# Autodesk Inventor assembly: SPE0V1 Ensamble General
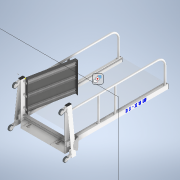
[picture p0: Inventor's stored thumbnail of the model, 180x180]
Saved by Autodesk Inventor 2021.2 (Build 252289000, 289)
## iProperties
Created: 2026-05-12
Part Number: SPE0V1 Ensamble General
Document SubType Name: Assembly
Designer: nelso
Author: nelso
## Documents named in this file (19)
- C:\Users\nelso\Desktop\Soporte-Paciente-Espinografia\Workspace\SPE0V1 Ensamble General.iam
- C:\Users\nelso\Desktop\Soporte-Paciente-Espinografia\Workspace\SP25V1 Acrilico.ipt
- C:\Users\nelso\Desktop\Soporte-Paciente-Espinografia\Workspace\SPE1V1 Estructura.iam
- C:\Users\nelso\Desktop\Soporte-Paciente-Espinografia\Workspace\SPE2V1 Baranda.iam
- C:\Users\nelso\Desktop\Soporte-Paciente-Espinografia\Workspace\DIN933M8X1.25L20C.ipt
- C:\Users\nelso\Desktop\Soporte-Paciente-Espinografia\Workspace\DIN125-A8,4C.ipt
- C:\Users\nelso\Desktop\Soporte-Paciente-Espinografia\Workspace\Logo.ipt
- C:\Users\nelso\Desktop\Soporte-Paciente-Espinografia\Workspace\SP28V1 Seguro Acrilico.ipt
- C:\Users\nelso\Desktop\Soporte-Paciente-Espinografia\Workspace\SP26V1 Base Chapa.ipt
- C:\Users\nelso\Desktop\Soporte-Paciente-Espinografia\Workspace\SP32V1 Refuerzo.ipt
- C:\Users\nelso\Desktop\Soporte-Paciente-Espinografia\Workspace\SPE31V1 Bisagra.iam
- C:\Users\nelso\Desktop\Soporte-Paciente-Espinografia\Workspace\SP39V1 Chapa Acrilico.ipt
- C:\Users\nelso\Desktop\Soporte-Paciente-Espinografia\Workspace\ISO7380M4X0.8L16I.ipt
- C:\Users\nelso\Desktop\Soporte-Paciente-Espinografia\Workspace\DIN555-5M4X0.8I.ipt
- C:\Users\nelso\Desktop\Soporte-Paciente-Espinografia\Workspace\SPE37V1 Cierre Superior.iam
- C:\Users\nelso\Desktop\Soporte-Paciente-Espinografia\Workspace\DIN125A4C.ipt
- C:\Users\nelso\Desktop\Soporte-Paciente-Espinografia\Workspace\DIN 555A5C.ipt
- C:\Users\nelso\Desktop\Soporte-Paciente-Espinografia\Workspace\DIN125-A6C.ipt
- C:\Users\nelso\Desktop\Soporte-Paciente-Espinografia\Workspace\DIN912-M6X1L16P.ipt
## Components (140 placed, 18 different names)
1. SP26V1 Base Chapa:1 — Mate:343, Mate:344, Mate:345, Mate:346, Mate:347, Mate:348, Mate:350, Mate:351, Mate:352, Mate:353, Mate:354, Flush:49, Flush:50, Flush:51, Angle:1, Mate:500, Mate:501, Mate:502, Mate:503, Mate:504, Mate:505
2. SP25V1 Acrilico:1 — Mate:179, Mate:180, Flush:19, Flush:20, Mate:262, Mate:355, Mate:356, Mate:357, Flush:52, Flush:53
3. SPE1V1 Estructura:1 [sub-assembly] — Coincidencia:100, Coincidencia:101, Coincidencia:102, Coincidencia:117, Nivelación:14, Nivelación:15, Mate:235, Mate:236, Mate:237, Flush:40, Mate:239, Mate:240, Mate:241, Flush:42, Mate:324, Mate:325, Flush:47, Flush:48, Mate:331, Mate:332, Mate:333, Mate:337, Mate:338, Mate:339, Mate:340, Mate:341, Mate:342, Angle:1, Flush:52, Mate:451, Mate:513, Mate:514, Mate:516, Mate:517, Mate:524, Mate:526
4. SPE2V1 Baranda:2 [sub-assembly] — Coincidencia:100, Coincidencia:101, Coincidencia:102, Coincidencia:109, Coincidencia:110, Coincidencia:111, Coincidencia:112, Mate:134, Mate:135, Mate:136, Mate:137, Mate:138, Mate:139, Mate:140, Mate:141, Mate:142, Mate:143, Mate:144, Mate:145, Mate:168, Mate:169, Mate:170, Mate:171, Mate:172, Mate:173
5. SPE2V1 Baranda:3 [sub-assembly] — Mate:118, Mate:119, Mate:120, Mate:121, Mate:122, Mate:123, Mate:124, Mate:125, Mate:126, Mate:127, Mate:128, Mate:129, Mate:130, Mate:131, Mate:132, Mate:133, Mate:147, Mate:149, Mate:156, Mate:157, Mate:158, Mate:159, Mate:160, Mate:161, Mate:235, Mate:236
6. DIN933M8X1.25L20C:1 — Coincidencia:113, Coincidencia:114
7. DIN125-A8,4C:1 — Coincidencia:109, Coincidencia:110, Coincidencia:115, Coincidencia:116
8. DIN125-A8,4C:2 — Coincidencia:111, Coincidencia:112, Coincidencia:113, Coincidencia:114
9. DIN933M8X1.25L20C:2 — Coincidencia:115, Coincidencia:116
10. Logo:1 — Coincidencia:117, Nivelación:14, Nivelación:15
11. DIN125-A8,4C:3 — Mate:144, Mate:145, Mate:162
12. DIN125-A8,4C:4 — Mate:142, Mate:143, Mate:163
13. DIN125-A8,4C:5 — Mate:140, Mate:141, Mate:164
14. DIN125-A8,4C:6 — Mate:138, Mate:139, Mate:165
15. DIN125-A8,4C:7 — Mate:135, Mate:136, Mate:167
16. DIN125-A8,4C:8 — Mate:134, Mate:137, Mate:166
17. DIN125-A8,4C:9 — Mate:130, Mate:132, Mate:155
18. DIN125-A8,4C:10 — Mate:131, Mate:133, Mate:154
19. DIN125-A8,4C:11 — Mate:128, Mate:129, Mate:153
20. DIN125-A8,4C:12 — Mate:126, Mate:127, Mate:152
21. DIN125-A8,4C:13 — Mate:122, Mate:123, Mate:150
22. DIN125-A8,4C:14 — Mate:124, Mate:125, Mate:151
23. DIN125-A8,4C:15 — Mate:120, Mate:121, Mate:148
24. DIN125-A8,4C:16 — Mate:118, Mate:119, Mate:146
25. DIN933M8X1.25L20C:3 — Mate:162, Mate:168
26. DIN933M8X1.25L20C:4 — Mate:163, Mate:169
27. DIN933M8X1.25L20C:5 — Mate:164, Mate:170
28. DIN933M8X1.25L20C:6 — Mate:165, Mate:171
29. DIN933M8X1.25L20C:7 — Mate:166, Mate:172
30. DIN933M8X1.25L20C:8 — Mate:167, Mate:173
31. DIN933M8X1.25L20C:9 — Mate:155, Mate:156
32. DIN933M8X1.25L20C:10 — Mate:154, Mate:157
33. DIN933M8X1.25L20C:11 — Mate:153, Mate:159
34. DIN933M8X1.25L20C:12 — Mate:152, Mate:158
35. DIN933M8X1.25L20C:13 — Mate:151, Mate:160
36. DIN933M8X1.25L20C:14 — Mate:150, Mate:161, Mate:237
37. DIN933M8X1.25L20C:15 — Mate:148, Mate:149
38. DIN933M8X1.25L20C:16 — Mate:146, Mate:147
39. SP28V1 Seguro Acrilico:1 — Mate:179, Flush:19, Mate:199, Mate:200, Mate:201, Mate:202, Mate:203, Mate:204, Mate:205, Mate:206, Mate:207, Mate:217, Mate:218, Mate:219, Mate:220, Mate:221, Mate:222, Mate:223, Mate:224, Mate:225, Flush:53
40. SP28V1 Seguro Acrilico:2 — Mate:180, Flush:20, Mate:208, Mate:209, Mate:210, Mate:211, Mate:212, Mate:213, Mate:214, Mate:215, Mate:216, Mate:227, Mate:228, Mate:229, Mate:230, Mate:231, Mate:233, Flush:40, Flush:42, Mate:448, Mate:449, Mate:450
41. ISO7380M4X0.8L16I:1 — Mate:199, Mate:217, Mate:358, Mate:411
42. ISO7380M4X0.8L16I:2 — Mate:200, Mate:218, Mate:359, Mate:410
43. ISO7380M4X0.8L16I:3 — Mate:201, Mate:219, Mate:360, Mate:409
44. ISO7380M4X0.8L16I:4 — Mate:202, Mate:220, Mate:361, Mate:408
45. ISO7380M4X0.8L16I:5 — Mate:203, Mate:221, Mate:362, Mate:407
46. ISO7380M4X0.8L16I:6 — Mate:204, Mate:222, Mate:363, Mate:406
47. ISO7380M4X0.8L16I:7 — Mate:205, Mate:223, Mate:364, Mate:405
48. ISO7380M4X0.8L16I:8 — Mate:206, Mate:224, Mate:365, Mate:404
49. ISO7380M4X0.8L16I:9 — Mate:207, Mate:225, Mate:366, Mate:403
50. ISO7380M4X0.8L16I:10 — Mate:208, Mate:262, Mate:367, Mate:394, Mate:449
51. ISO7380M4X0.8L16I:11 — Mate:209, Mate:233, Mate:368, Mate:395
52. ISO7380M4X0.8L16I:12 — Mate:210, Mate:369, Mate:396, Mate:450
53. ISO7380M4X0.8L16I:13 — Mate:211, Mate:231, Mate:370, Mate:397
54. ISO7380M4X0.8L16I:14 — Mate:212, Mate:230, Mate:371, Mate:398
55. ISO7380M4X0.8L16I:15 — Mate:214, Mate:228, Mate:373, Mate:400
56. ISO7380M4X0.8L16I:16 — Mate:215, Mate:227, Mate:374, Mate:402
57. ISO7380M4X0.8L16I:17 — Mate:216, Mate:375, Mate:401, Mate:448
58. ISO7380M4X0.8L16I:18 — Mate:213, Mate:229, Mate:372, Mate:399
59. SP32V1 Refuerzo:1 — Mate:351, Mate:354, Flush:50
60. SP32V1 Refuerzo:2 — Mate:348, Mate:353, Flush:49
61. SP32V1 Refuerzo:3 — Mate:350, Mate:352, Flush:51
62. SPE31V1 Bisagra:1 [sub-assembly] — Mate:333, Mate:341, Mate:342, Mate:345, Mate:347, Mate:468, Mate:469, Mate:470, Mate:471, Mate:472, Mate:473, Mate:474, Mate:475
63. SPE31V1 Bisagra:2 [sub-assembly] — Mate:331, Mate:337, Mate:338, Mate:344, Mate:346, Mate:452, Mate:453, Mate:454, Mate:455, Mate:456, Mate:457, Mate:458, Mate:459
64. SPE31V1 Bisagra:3 [sub-assembly] — Mate:332, Mate:339, Mate:340, Mate:343, Mate:460, Mate:461, Mate:462, Mate:463, Mate:464, Mate:465, Mate:466, Mate:467
65. SP39V1 Chapa Acrilico:1 — Mate:325, Flush:47, Mate:355, Mate:430, Mate:432, Mate:434, Mate:436, Mate:438, Mate:440, Mate:442, Mate:444, Mate:446
66. SP39V1 Chapa Acrilico:2 — Mate:324, Flush:48, Mate:357, Mate:412, Mate:414, Mate:416, Mate:418, Mate:420, Mate:422, Mate:424, Mate:426, Mate:428
67. DIN555-5M4X0.8I:1 — Mate:358, Mate:413
68. DIN555-5M4X0.8I:2 — Mate:359, Mate:415
69. DIN555-5M4X0.8I:3 — Mate:360, Mate:417
70. DIN555-5M4X0.8I:4 — Mate:361, Mate:419
71. DIN555-5M4X0.8I:5 — Mate:362, Mate:421
72. DIN555-5M4X0.8I:6 — Mate:363, Mate:423
73. DIN555-5M4X0.8I:7 — Mate:364, Mate:425
74. DIN555-5M4X0.8I:8 — Mate:365, Mate:427
75. DIN555-5M4X0.8I:9 — Mate:366, Mate:429
76. DIN555-5M4X0.8I:10 — Mate:367, Mate:447
77. DIN555-5M4X0.8I:11 — Mate:368, Mate:445
78. DIN555-5M4X0.8I:12 — Mate:369, Mate:443
79. DIN555-5M4X0.8I:13 — Mate:370, Mate:441
80. DIN555-5M4X0.8I:14 — Mate:371, Mate:439
81. DIN555-5M4X0.8I:15 — Mate:372, Mate:437
82. DIN555-5M4X0.8I:16 — Mate:373, Mate:435
83. DIN555-5M4X0.8I:17 — Mate:374, Mate:433
84. DIN555-5M4X0.8I:18 — Mate:375, Mate:431
85. DIN125A4C:2 — Mate:411, Mate:412, Mate:413
86. DIN125A4C:3 — Mate:410, Mate:414, Mate:415
87. DIN125A4C:4 — Mate:409, Mate:416, Mate:417
88. DIN125A4C:5 — Mate:408, Mate:418, Mate:419
89. DIN125A4C:6 — Mate:407, Mate:420, Mate:421
90. DIN125A4C:7 — Mate:406, Mate:422, Mate:423
91. DIN125A4C:8 — Mate:405, Mate:424, Mate:425
92. DIN125A4C:9 — Mate:404, Mate:426, Mate:427
93. DIN125A4C:10 — Mate:403, Mate:428, Mate:429
94. DIN125A4C:11 — Mate:402, Mate:432, Mate:433
95. DIN125A4C:12 — Mate:401, Mate:430, Mate:431
96. DIN125A4C:13 — Mate:400, Mate:434, Mate:435
97. DIN125A4C:14 — Mate:399, Mate:436, Mate:437
98. DIN125A4C:15 — Mate:398, Mate:438, Mate:439
99. DIN125A4C:16 — Mate:397, Mate:440, Mate:441
100. DIN125A4C:17 — Mate:396, Mate:442, Mate:443
101. DIN125A4C:18 — Mate:395, Mate:444, Mate:445
102. DIN125A4C:19 — Mate:394, Mate:446, Mate:447
103. SPE37V1 Cierre Superior:1 [sub-assembly] — Mate:451
104. DIN912-M6X1L16P:2 — Mate:452, Mate:454, Mate:522
105. DIN912-M6X1L16P:3 — Mate:453, Mate:455, Mate:523, Mate:525
106. DIN912-M6X1L16P:4 — Mate:456, Mate:457, Mate:506
107. DIN912-M6X1L16P:5 — Mate:458, Mate:459, Mate:507
108. DIN912-M6X1L16P:6 — Mate:460, Mate:464, Mate:518
109. DIN912-M6X1L16P:7 — Mate:462, Mate:466, Mate:508
110. DIN912-M6X1L16P:8 — Mate:461, Mate:465, Mate:519
111. DIN912-M6X1L16P:9 — Mate:463, Mate:467, Mate:509
112. DIN912-M6X1L16P:10 — Mate:469, Mate:473, Mate:521
113. DIN912-M6X1L16P:11 — Mate:468, Mate:472, Mate:520
114. DIN912-M6X1L16P:12 — Mate:470, Mate:474, Mate:510
115. DIN912-M6X1L16P:13 — Mate:471, Mate:475, Mate:511
116. DIN 555A5C:1 — Mate:476, Mate:488, Mate:519
117. DIN 555A5C:2 — Mate:477, Mate:489, Mate:506
118. DIN 555A5C:3 — Mate:478, Mate:523
119. DIN 555A5C:4 — Mate:479, Mate:491, Mate:509
120. DIN 555A5C:5 — Mate:480, Mate:492, Mate:518
121. DIN 555A5C:6 — Mate:481, Mate:493, Mate:508
122. DIN 555A5C:7 — Mate:482, Mate:494, Mate:521
123. DIN 555A5C:8 — Mate:483, Mate:495, Mate:510
124. DIN 555A5C:9 — Mate:485, Mate:497, Mate:522
125. DIN 555A5C:10 — Mate:484, Mate:496, Mate:507
126. DIN 555A5C:11 — Mate:486, Mate:498, Mate:511
127. DIN 555A5C:12 — Mate:487, Mate:499, Mate:520
128. DIN125-A6C:1 — Mate:476, Mate:488, Mate:513
129. DIN125-A6C:2 — Mate:477, Mate:489, Mate:500
130. DIN125-A6C:3 — Mate:478, Mate:524, Mate:525
131. DIN125-A6C:4 — Mate:479, Mate:491, Mate:502
132. DIN125-A6C:5 — Mate:480, Mate:492, Mate:514
133. DIN125-A6C:6 — Mate:481, Mate:493, Mate:503
134. DIN125-A6C:7 — Mate:482, Mate:494, Mate:517
135. DIN125-A6C:8 — Mate:483, Mate:495, Mate:504
136. DIN125-A6C:9 — Mate:484, Mate:496, Mate:501
137. DIN125-A6C:10 — Mate:485, Mate:497, Mate:526
138. DIN125-A6C:11 — Mate:486, Mate:498, Mate:505
139. DIN125-A6C:12 — Mate:487, Mate:499, Mate:516
140. DIN912-M6X1L16P:1
## Relationships (297: Mate 283, Flush 13, Angle 1)
- Coincidencia:100 [Mate]: SPE1V1 Estructura:1 ↔ SPE2V1 Baranda:2
- Coincidencia:101 [Mate]: SPE1V1 Estructura:1 ↔ SPE2V1 Baranda:2
- Coincidencia:102 [Mate]: SPE1V1 Estructura:1 ↔ SPE2V1 Baranda:2
- Coincidencia:109 [Mate]: SPE2V1 Baranda:2 ↔ DIN125-A8,4C:1
- Coincidencia:110 [Mate]: SPE2V1 Baranda:2 ↔ DIN125-A8,4C:1
- Coincidencia:111 [Mate]: SPE2V1 Baranda:2 ↔ DIN125-A8,4C:2
- Coincidencia:112 [Mate]: SPE2V1 Baranda:2 ↔ DIN125-A8,4C:2
- Coincidencia:113 [Mate]: DIN933M8X1.25L20C:1 ↔ DIN125-A8,4C:2
- Coincidencia:114 [Mate]: DIN933M8X1.25L20C:1 ↔ DIN125-A8,4C:2
- Coincidencia:115 [Mate]: DIN125-A8,4C:1 ↔ DIN933M8X1.25L20C:2
- Coincidencia:116 [Mate]: DIN125-A8,4C:1 ↔ DIN933M8X1.25L20C:2
- Coincidencia:117 [Mate]: SPE1V1 Estructura:1 ↔ Logo:1
- Nivelación:14 [Flush] (10 mm): SPE1V1 Estructura:1 ↔ Logo:1
- Nivelación:15 [Flush] (400 mm): SPE1V1 Estructura:1 ↔ Logo:1
- Mate:118: SPE2V1 Baranda:3 ↔ DIN125-A8,4C:16
- Mate:119: SPE2V1 Baranda:3 ↔ DIN125-A8,4C:16
- Mate:120: SPE2V1 Baranda:3 ↔ DIN125-A8,4C:15
- Mate:121: SPE2V1 Baranda:3 ↔ DIN125-A8,4C:15
- Mate:122: SPE2V1 Baranda:3 ↔ DIN125-A8,4C:13
- Mate:123: SPE2V1 Baranda:3 ↔ DIN125-A8,4C:13
- Mate:124: SPE2V1 Baranda:3 ↔ DIN125-A8,4C:14
- Mate:125: SPE2V1 Baranda:3 ↔ DIN125-A8,4C:14
- Mate:126: SPE2V1 Baranda:3 ↔ DIN125-A8,4C:12
- Mate:127: SPE2V1 Baranda:3 ↔ DIN125-A8,4C:12
- Mate:128: SPE2V1 Baranda:3 ↔ DIN125-A8,4C:11
- Mate:129: SPE2V1 Baranda:3 ↔ DIN125-A8,4C:11
- Mate:130: SPE2V1 Baranda:3 ↔ DIN125-A8,4C:9
- Mate:131: SPE2V1 Baranda:3 ↔ DIN125-A8,4C:10
- Mate:132: SPE2V1 Baranda:3 ↔ DIN125-A8,4C:9
- Mate:133: SPE2V1 Baranda:3 ↔ DIN125-A8,4C:10
- Mate:134: SPE2V1 Baranda:2 ↔ DIN125-A8,4C:8
- Mate:135: SPE2V1 Baranda:2 ↔ DIN125-A8,4C:7
- Mate:136: SPE2V1 Baranda:2 ↔ DIN125-A8,4C:7
- Mate:137: SPE2V1 Baranda:2 ↔ DIN125-A8,4C:8
- Mate:138: SPE2V1 Baranda:2 ↔ DIN125-A8,4C:6
- Mate:139: SPE2V1 Baranda:2 ↔ DIN125-A8,4C:6
- Mate:140: SPE2V1 Baranda:2 ↔ DIN125-A8,4C:5
- Mate:141: SPE2V1 Baranda:2 ↔ DIN125-A8,4C:5
- Mate:142: SPE2V1 Baranda:2 ↔ DIN125-A8,4C:4
- Mate:143: SPE2V1 Baranda:2 ↔ DIN125-A8,4C:4
- Mate:144: SPE2V1 Baranda:2 ↔ DIN125-A8,4C:3
- Mate:145: SPE2V1 Baranda:2 ↔ DIN125-A8,4C:3
- Mate:146: DIN125-A8,4C:16 ↔ DIN933M8X1.25L20C:16
- Mate:147: SPE2V1 Baranda:3 ↔ DIN933M8X1.25L20C:16
- Mate:148: DIN125-A8,4C:15 ↔ DIN933M8X1.25L20C:15
- Mate:149: SPE2V1 Baranda:3 ↔ DIN933M8X1.25L20C:15
- Mate:150: DIN125-A8,4C:13 ↔ DIN933M8X1.25L20C:14
- Mate:151: DIN125-A8,4C:14 ↔ DIN933M8X1.25L20C:13
- Mate:152: DIN125-A8,4C:12 ↔ DIN933M8X1.25L20C:12
- Mate:153: DIN125-A8,4C:11 ↔ DIN933M8X1.25L20C:11
- Mate:154: DIN125-A8,4C:10 ↔ DIN933M8X1.25L20C:10
- Mate:155: DIN125-A8,4C:9 ↔ DIN933M8X1.25L20C:9
- Mate:156: SPE2V1 Baranda:3 ↔ DIN933M8X1.25L20C:9
- Mate:157: SPE2V1 Baranda:3 ↔ DIN933M8X1.25L20C:10
- Mate:158: SPE2V1 Baranda:3 ↔ DIN933M8X1.25L20C:12
- Mate:159: SPE2V1 Baranda:3 ↔ DIN933M8X1.25L20C:11
- Mate:160: SPE2V1 Baranda:3 ↔ DIN933M8X1.25L20C:13
- Mate:161: SPE2V1 Baranda:3 ↔ DIN933M8X1.25L20C:14
- Mate:162: DIN125-A8,4C:3 ↔ DIN933M8X1.25L20C:3
- Mate:163: DIN125-A8,4C:4 ↔ DIN933M8X1.25L20C:4
- Mate:164: DIN125-A8,4C:5 ↔ DIN933M8X1.25L20C:5
- Mate:165: DIN125-A8,4C:6 ↔ DIN933M8X1.25L20C:6
- Mate:166: DIN125-A8,4C:8 ↔ DIN933M8X1.25L20C:7
- Mate:167: DIN125-A8,4C:7 ↔ DIN933M8X1.25L20C:8
- Mate:168: SPE2V1 Baranda:2 ↔ DIN933M8X1.25L20C:3
- Mate:169: SPE2V1 Baranda:2 ↔ DIN933M8X1.25L20C:4
- Mate:170: SPE2V1 Baranda:2 ↔ DIN933M8X1.25L20C:5
- Mate:171: SPE2V1 Baranda:2 ↔ DIN933M8X1.25L20C:6
- Mate:172: SPE2V1 Baranda:2 ↔ DIN933M8X1.25L20C:7
- Mate:173: SPE2V1 Baranda:2 ↔ DIN933M8X1.25L20C:8
- Mate:179: SP25V1 Acrilico:1 ↔ SP28V1 Seguro Acrilico:1
- Mate:180: SP25V1 Acrilico:1 ↔ SP28V1 Seguro Acrilico:2
- Flush:19: SP25V1 Acrilico:1 ↔ SP28V1 Seguro Acrilico:1
- Flush:20: SP25V1 Acrilico:1 ↔ SP28V1 Seguro Acrilico:2
- Mate:199: SP28V1 Seguro Acrilico:1 ↔ ISO7380M4X0.8L16I:1
- Mate:200: SP28V1 Seguro Acrilico:1 ↔ ISO7380M4X0.8L16I:2
- Mate:201: SP28V1 Seguro Acrilico:1 ↔ ISO7380M4X0.8L16I:3
- Mate:202: SP28V1 Seguro Acrilico:1 ↔ ISO7380M4X0.8L16I:4
- Mate:203: SP28V1 Seguro Acrilico:1 ↔ ISO7380M4X0.8L16I:5
- Mate:204: SP28V1 Seguro Acrilico:1 ↔ ISO7380M4X0.8L16I:6
- Mate:205: SP28V1 Seguro Acrilico:1 ↔ ISO7380M4X0.8L16I:7
- Mate:206: SP28V1 Seguro Acrilico:1 ↔ ISO7380M4X0.8L16I:8
- Mate:207: SP28V1 Seguro Acrilico:1 ↔ ISO7380M4X0.8L16I:9
- Mate:208: SP28V1 Seguro Acrilico:2 ↔ ISO7380M4X0.8L16I:10
- Mate:209: SP28V1 Seguro Acrilico:2 ↔ ISO7380M4X0.8L16I:11
- Mate:210: SP28V1 Seguro Acrilico:2 ↔ ISO7380M4X0.8L16I:12
- Mate:211: SP28V1 Seguro Acrilico:2 ↔ ISO7380M4X0.8L16I:13
- Mate:212: SP28V1 Seguro Acrilico:2 ↔ ISO7380M4X0.8L16I:14
- Mate:213: SP28V1 Seguro Acrilico:2 ↔ ISO7380M4X0.8L16I:18
- Mate:214: SP28V1 Seguro Acrilico:2 ↔ ISO7380M4X0.8L16I:15
- Mate:215: SP28V1 Seguro Acrilico:2 ↔ ISO7380M4X0.8L16I:16
- Mate:216: SP28V1 Seguro Acrilico:2 ↔ ISO7380M4X0.8L16I:17
- Mate:217: SP28V1 Seguro Acrilico:1 ↔ ISO7380M4X0.8L16I:1
- Mate:218: SP28V1 Seguro Acrilico:1 ↔ ISO7380M4X0.8L16I:2
- Mate:219: SP28V1 Seguro Acrilico:1 ↔ ISO7380M4X0.8L16I:3
- Mate:220: SP28V1 Seguro Acrilico:1 ↔ ISO7380M4X0.8L16I:4
- Mate:221: SP28V1 Seguro Acrilico:1 ↔ ISO7380M4X0.8L16I:5
- Mate:222: SP28V1 Seguro Acrilico:1 ↔ ISO7380M4X0.8L16I:6
- Mate:223: SP28V1 Seguro Acrilico:1 ↔ ISO7380M4X0.8L16I:7
- Mate:224: SP28V1 Seguro Acrilico:1 ↔ ISO7380M4X0.8L16I:8
- Mate:225: SP28V1 Seguro Acrilico:1 ↔ ISO7380M4X0.8L16I:9
- Mate:227: SP28V1 Seguro Acrilico:2 ↔ ISO7380M4X0.8L16I:16
- Mate:228: SP28V1 Seguro Acrilico:2 ↔ ISO7380M4X0.8L16I:15
- Mate:229: SP28V1 Seguro Acrilico:2 ↔ ISO7380M4X0.8L16I:18
- Mate:230: SP28V1 Seguro Acrilico:2 ↔ ISO7380M4X0.8L16I:14
- Mate:231: SP28V1 Seguro Acrilico:2 ↔ ISO7380M4X0.8L16I:13
- Mate:233: SP28V1 Seguro Acrilico:2 ↔ ISO7380M4X0.8L16I:11
- Mate:235: SPE1V1 Estructura:1 ↔ SPE2V1 Baranda:3
- Mate:236: SPE1V1 Estructura:1 ↔ SPE2V1 Baranda:3
- Mate:237: SPE1V1 Estructura:1 ↔ DIN933M8X1.25L20C:14
- Flush:40: SPE1V1 Estructura:1 ↔ SP28V1 Seguro Acrilico:2
- Mate:239: SPE1V1 Estructura:1
- Mate:240: SPE1V1 Estructura:1
- Mate:241: SPE1V1 Estructura:1
- Flush:42: SPE1V1 Estructura:1 ↔ SP28V1 Seguro Acrilico:2
- Mate:262: SP25V1 Acrilico:1 ↔ ISO7380M4X0.8L16I:10
- Mate:324: SPE1V1 Estructura:1 ↔ SP39V1 Chapa Acrilico:2
- Mate:325: SPE1V1 Estructura:1 ↔ SP39V1 Chapa Acrilico:1
- Flush:47: SPE1V1 Estructura:1 ↔ SP39V1 Chapa Acrilico:1
- Flush:48: SPE1V1 Estructura:1 ↔ SP39V1 Chapa Acrilico:2
- Mate:331: SPE1V1 Estructura:1 ↔ SPE31V1 Bisagra:2
- Mate:332: SPE1V1 Estructura:1 ↔ SPE31V1 Bisagra:3
- Mate:333: SPE1V1 Estructura:1 ↔ SPE31V1 Bisagra:1
- Mate:337: SPE1V1 Estructura:1 ↔ SPE31V1 Bisagra:2
- Mate:338: SPE1V1 Estructura:1 ↔ SPE31V1 Bisagra:2
- Mate:339: SPE1V1 Estructura:1 ↔ SPE31V1 Bisagra:3
- Mate:340: SPE1V1 Estructura:1 ↔ SPE31V1 Bisagra:3
- Mate:341: SPE1V1 Estructura:1 ↔ SPE31V1 Bisagra:1
- Mate:342: SPE1V1 Estructura:1 ↔ SPE31V1 Bisagra:1
- Mate:343: SP26V1 Base Chapa:1 ↔ SPE31V1 Bisagra:3
- Mate:344: SP26V1 Base Chapa:1 ↔ SPE31V1 Bisagra:2
- Mate:345: SP26V1 Base Chapa:1 ↔ SPE31V1 Bisagra:1
- Mate:346: SP26V1 Base Chapa:1 ↔ SPE31V1 Bisagra:2
- Mate:347: SP26V1 Base Chapa:1 ↔ SPE31V1 Bisagra:1
- Mate:348: SP26V1 Base Chapa:1 ↔ SP32V1 Refuerzo:2
- Mate:350: SP26V1 Base Chapa:1 ↔ SP32V1 Refuerzo:3
- Mate:351: SP26V1 Base Chapa:1 ↔ SP32V1 Refuerzo:1
- Mate:352: SP26V1 Base Chapa:1 ↔ SP32V1 Refuerzo:3
- Mate:353: SP26V1 Base Chapa:1 ↔ SP32V1 Refuerzo:2
- Mate:354: SP26V1 Base Chapa:1 ↔ SP32V1 Refuerzo:1
- Flush:49: SP26V1 Base Chapa:1 ↔ SP32V1 Refuerzo:2
- Flush:50: SP26V1 Base Chapa:1 ↔ SP32V1 Refuerzo:1
- Flush:51: SP26V1 Base Chapa:1 ↔ SP32V1 Refuerzo:3
- Angle:1 (0 deg): SP26V1 Base Chapa:1 ↔ SPE1V1 Estructura:1
- Mate:355: SP25V1 Acrilico:1 ↔ SP39V1 Chapa Acrilico:1
- Mate:356: SP25V1 Acrilico:1
- Mate:357: SP25V1 Acrilico:1 ↔ SP39V1 Chapa Acrilico:2
- Flush:52: SP25V1 Acrilico:1 ↔ SPE1V1 Estructura:1
- Flush:53: SP25V1 Acrilico:1 ↔ SP28V1 Seguro Acrilico:1
- Mate:358: ISO7380M4X0.8L16I:1 ↔ DIN555-5M4X0.8I:1
- Mate:359: ISO7380M4X0.8L16I:2 ↔ DIN555-5M4X0.8I:2
- Mate:360: ISO7380M4X0.8L16I:3 ↔ DIN555-5M4X0.8I:3
- Mate:361: ISO7380M4X0.8L16I:4 ↔ DIN555-5M4X0.8I:4
- Mate:362: ISO7380M4X0.8L16I:5 ↔ DIN555-5M4X0.8I:5
- Mate:363: ISO7380M4X0.8L16I:6 ↔ DIN555-5M4X0.8I:6
- Mate:364: ISO7380M4X0.8L16I:7 ↔ DIN555-5M4X0.8I:7
- Mate:365: ISO7380M4X0.8L16I:8 ↔ DIN555-5M4X0.8I:8
- Mate:366: ISO7380M4X0.8L16I:9 ↔ DIN555-5M4X0.8I:9
- Mate:367: ISO7380M4X0.8L16I:10 ↔ DIN555-5M4X0.8I:10
- Mate:368: ISO7380M4X0.8L16I:11 ↔ DIN555-5M4X0.8I:11
- Mate:369: ISO7380M4X0.8L16I:12 ↔ DIN555-5M4X0.8I:12
- Mate:370: ISO7380M4X0.8L16I:13 ↔ DIN555-5M4X0.8I:13
- Mate:371: ISO7380M4X0.8L16I:14 ↔ DIN555-5M4X0.8I:14
- Mate:372: ISO7380M4X0.8L16I:18 ↔ DIN555-5M4X0.8I:15
- Mate:373: ISO7380M4X0.8L16I:15 ↔ DIN555-5M4X0.8I:16
- Mate:374: ISO7380M4X0.8L16I:16 ↔ DIN555-5M4X0.8I:17
- Mate:375: ISO7380M4X0.8L16I:17 ↔ DIN555-5M4X0.8I:18
- Mate:394: ISO7380M4X0.8L16I:10 ↔ DIN125A4C:19
- Mate:395: ISO7380M4X0.8L16I:11 ↔ DIN125A4C:18
- Mate:396: ISO7380M4X0.8L16I:12 ↔ DIN125A4C:17
- Mate:397: ISO7380M4X0.8L16I:13 ↔ DIN125A4C:16
- Mate:398: ISO7380M4X0.8L16I:14 ↔ DIN125A4C:15
- Mate:399: ISO7380M4X0.8L16I:18 ↔ DIN125A4C:14
- Mate:400: ISO7380M4X0.8L16I:15 ↔ DIN125A4C:13
- Mate:401: ISO7380M4X0.8L16I:17 ↔ DIN125A4C:12
- Mate:402: ISO7380M4X0.8L16I:16 ↔ DIN125A4C:11
- Mate:403: ISO7380M4X0.8L16I:9 ↔ DIN125A4C:10
- Mate:404: ISO7380M4X0.8L16I:8 ↔ DIN125A4C:9
- Mate:405: ISO7380M4X0.8L16I:7 ↔ DIN125A4C:8
- Mate:406: ISO7380M4X0.8L16I:6 ↔ DIN125A4C:7
- Mate:407: ISO7380M4X0.8L16I:5 ↔ DIN125A4C:6
- Mate:408: ISO7380M4X0.8L16I:4 ↔ DIN125A4C:5
- Mate:409: ISO7380M4X0.8L16I:3 ↔ DIN125A4C:4
- Mate:410: ISO7380M4X0.8L16I:2 ↔ DIN125A4C:3
- Mate:411: ISO7380M4X0.8L16I:1 ↔ DIN125A4C:2
- Mate:412: SP39V1 Chapa Acrilico:2 ↔ DIN125A4C:2
- Mate:413: DIN555-5M4X0.8I:1 ↔ DIN125A4C:2
- Mate:414: SP39V1 Chapa Acrilico:2 ↔ DIN125A4C:3
- Mate:415: DIN555-5M4X0.8I:2 ↔ DIN125A4C:3
- Mate:416: SP39V1 Chapa Acrilico:2 ↔ DIN125A4C:4
- Mate:417: DIN555-5M4X0.8I:3 ↔ DIN125A4C:4
- Mate:418: SP39V1 Chapa Acrilico:2 ↔ DIN125A4C:5
- Mate:419: DIN555-5M4X0.8I:4 ↔ DIN125A4C:5
- Mate:420: SP39V1 Chapa Acrilico:2 ↔ DIN125A4C:6
- Mate:421: DIN555-5M4X0.8I:5 ↔ DIN125A4C:6
- Mate:422: SP39V1 Chapa Acrilico:2 ↔ DIN125A4C:7
- Mate:423: DIN555-5M4X0.8I:6 ↔ DIN125A4C:7
- Mate:424: SP39V1 Chapa Acrilico:2 ↔ DIN125A4C:8
- Mate:425: DIN555-5M4X0.8I:7 ↔ DIN125A4C:8
- Mate:426: SP39V1 Chapa Acrilico:2 ↔ DIN125A4C:9
- Mate:427: DIN555-5M4X0.8I:8 ↔ DIN125A4C:9
- Mate:428: SP39V1 Chapa Acrilico:2 ↔ DIN125A4C:10
- Mate:429: DIN555-5M4X0.8I:9 ↔ DIN125A4C:10
- Mate:430: SP39V1 Chapa Acrilico:1 ↔ DIN125A4C:12
- Mate:431: DIN555-5M4X0.8I:18 ↔ DIN125A4C:12
- Mate:432: SP39V1 Chapa Acrilico:1 ↔ DIN125A4C:11
- Mate:433: DIN555-5M4X0.8I:17 ↔ DIN125A4C:11
- Mate:434: SP39V1 Chapa Acrilico:1 ↔ DIN125A4C:13
- Mate:435: DIN555-5M4X0.8I:16 ↔ DIN125A4C:13
- Mate:436: SP39V1 Chapa Acrilico:1 ↔ DIN125A4C:14
- Mate:437: DIN555-5M4X0.8I:15 ↔ DIN125A4C:14
- Mate:438: SP39V1 Chapa Acrilico:1 ↔ DIN125A4C:15
- Mate:439: DIN555-5M4X0.8I:14 ↔ DIN125A4C:15
- Mate:440: SP39V1 Chapa Acrilico:1 ↔ DIN125A4C:16
- Mate:441: DIN555-5M4X0.8I:13 ↔ DIN125A4C:16
- Mate:442: SP39V1 Chapa Acrilico:1 ↔ DIN125A4C:17
- Mate:443: DIN555-5M4X0.8I:12 ↔ DIN125A4C:17
- Mate:444: SP39V1 Chapa Acrilico:1 ↔ DIN125A4C:18
- Mate:445: DIN555-5M4X0.8I:11 ↔ DIN125A4C:18
- Mate:446: SP39V1 Chapa Acrilico:1 ↔ DIN125A4C:19
- Mate:447: DIN555-5M4X0.8I:10 ↔ DIN125A4C:19
- Mate:448: SP28V1 Seguro Acrilico:2 ↔ ISO7380M4X0.8L16I:17
- Mate:449: SP28V1 Seguro Acrilico:2 ↔ ISO7380M4X0.8L16I:10
- Mate:450: SP28V1 Seguro Acrilico:2 ↔ ISO7380M4X0.8L16I:12
- Mate:451 (2 mm): SPE1V1 Estructura:1 ↔ SPE37V1 Cierre Superior:1
- Mate:452: SPE31V1 Bisagra:2 ↔ DIN912-M6X1L16P:2
- Mate:453: SPE31V1 Bisagra:2 ↔ DIN912-M6X1L16P:3
- Mate:454: SPE31V1 Bisagra:2 ↔ DIN912-M6X1L16P:2
- Mate:455: SPE31V1 Bisagra:2 ↔ DIN912-M6X1L16P:3
- Mate:456: SPE31V1 Bisagra:2 ↔ DIN912-M6X1L16P:4
- Mate:457: SPE31V1 Bisagra:2 ↔ DIN912-M6X1L16P:4
- Mate:458: SPE31V1 Bisagra:2 ↔ DIN912-M6X1L16P:5
- Mate:459: SPE31V1 Bisagra:2 ↔ DIN912-M6X1L16P:5
- Mate:460: SPE31V1 Bisagra:3 ↔ DIN912-M6X1L16P:6
- Mate:461: SPE31V1 Bisagra:3 ↔ DIN912-M6X1L16P:8
- Mate:462: SPE31V1 Bisagra:3 ↔ DIN912-M6X1L16P:7
- Mate:463: SPE31V1 Bisagra:3 ↔ DIN912-M6X1L16P:9
- Mate:464: SPE31V1 Bisagra:3 ↔ DIN912-M6X1L16P:6
- Mate:465: SPE31V1 Bisagra:3 ↔ DIN912-M6X1L16P:8
- Mate:466: SPE31V1 Bisagra:3 ↔ DIN912-M6X1L16P:7
- Mate:467: SPE31V1 Bisagra:3 ↔ DIN912-M6X1L16P:9
- Mate:468: SPE31V1 Bisagra:1 ↔ DIN912-M6X1L16P:11
- Mate:469: SPE31V1 Bisagra:1 ↔ DIN912-M6X1L16P:10
- Mate:470: SPE31V1 Bisagra:1 ↔ DIN912-M6X1L16P:12
- Mate:471: SPE31V1 Bisagra:1 ↔ DIN912-M6X1L16P:13
- Mate:472: SPE31V1 Bisagra:1 ↔ DIN912-M6X1L16P:11
- Mate:473: SPE31V1 Bisagra:1 ↔ DIN912-M6X1L16P:10
- Mate:474: SPE31V1 Bisagra:1 ↔ DIN912-M6X1L16P:12
- Mate:475: SPE31V1 Bisagra:1 ↔ DIN912-M6X1L16P:13
- Mate:476: DIN 555A5C:1 ↔ DIN125-A6C:1
- Mate:477: DIN 555A5C:2 ↔ DIN125-A6C:2
- Mate:478: DIN 555A5C:3 ↔ DIN125-A6C:3
- Mate:479: DIN 555A5C:4 ↔ DIN125-A6C:4
- Mate:480: DIN 555A5C:5 ↔ DIN125-A6C:5
- Mate:481: DIN 555A5C:6 ↔ DIN125-A6C:6
- Mate:482: DIN 555A5C:7 ↔ DIN125-A6C:7
- Mate:483: DIN 555A5C:8 ↔ DIN125-A6C:8
- Mate:484: DIN 555A5C:10 ↔ DIN125-A6C:9
- Mate:485: DIN 555A5C:9 ↔ DIN125-A6C:10
- Mate:486: DIN 555A5C:11 ↔ DIN125-A6C:11
- Mate:487: DIN 555A5C:12 ↔ DIN125-A6C:12
- Mate:488: DIN 555A5C:1 ↔ DIN125-A6C:1
- Mate:489: DIN 555A5C:2 ↔ DIN125-A6C:2
- Mate:491: DIN 555A5C:4 ↔ DIN125-A6C:4
- Mate:492: DIN 555A5C:5 ↔ DIN125-A6C:5
- Mate:493: DIN 555A5C:6 ↔ DIN125-A6C:6
- Mate:494: DIN 555A5C:7 ↔ DIN125-A6C:7
- Mate:495: DIN 555A5C:8 ↔ DIN125-A6C:8
- Mate:496: DIN 555A5C:10 ↔ DIN125-A6C:9
- Mate:497: DIN 555A5C:9 ↔ DIN125-A6C:10
- Mate:498: DIN 555A5C:11 ↔ DIN125-A6C:11
- Mate:499: DIN 555A5C:12 ↔ DIN125-A6C:12
- Mate:500: SP26V1 Base Chapa:1 ↔ DIN125-A6C:2
- Mate:501: SP26V1 Base Chapa:1 ↔ DIN125-A6C:9
- Mate:502: SP26V1 Base Chapa:1 ↔ DIN125-A6C:4
- Mate:503: SP26V1 Base Chapa:1 ↔ DIN125-A6C:6
- Mate:504: SP26V1 Base Chapa:1 ↔ DIN125-A6C:8
- Mate:505: SP26V1 Base Chapa:1 ↔ DIN125-A6C:11
- Mate:506: DIN912-M6X1L16P:4 ↔ DIN 555A5C:2
- Mate:507: DIN912-M6X1L16P:5 ↔ DIN 555A5C:10
- Mate:508: DIN912-M6X1L16P:7 ↔ DIN 555A5C:6
- Mate:509: DIN912-M6X1L16P:9 ↔ DIN 555A5C:4
- Mate:510: DIN912-M6X1L16P:12 ↔ DIN 555A5C:8
- Mate:511: DIN912-M6X1L16P:13 ↔ DIN 555A5C:11
- Mate:513: SPE1V1 Estructura:1 ↔ DIN125-A6C:1
- Mate:514: SPE1V1 Estructura:1 ↔ DIN125-A6C:5
- Mate:516: SPE1V1 Estructura:1 ↔ DIN125-A6C:12
- Mate:517: SPE1V1 Estructura:1 ↔ DIN125-A6C:7
- Mate:518: DIN912-M6X1L16P:6 ↔ DIN 555A5C:5
- Mate:519: DIN912-M6X1L16P:8 ↔ DIN 555A5C:1
- Mate:520: DIN912-M6X1L16P:11 ↔ DIN 555A5C:12
- Mate:521: DIN912-M6X1L16P:10 ↔ DIN 555A5C:7
- Mate:522: DIN912-M6X1L16P:2 ↔ DIN 555A5C:9
- Mate:523: DIN912-M6X1L16P:3 ↔ DIN 555A5C:3
- Mate:524: SPE1V1 Estructura:1 ↔ DIN125-A6C:3
- Mate:525: DIN912-M6X1L16P:3 ↔ DIN125-A6C:3
- Mate:526: SPE1V1 Estructura:1 ↔ DIN125-A6C:10
